# Autodesk Inventor assembly: Sistema movimiento izquierdo
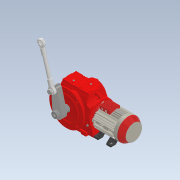
[picture p0: Inventor's stored thumbnail of the model, 180x180]
Saved by Autodesk Inventor 2021 (Build 250183000, 183)
## iProperties
Created: 2021-06-19
Part Number: Sistema movimiento izquierdo
Document SubType Name: Assembly
Designer: Andrés Holguín
Author: Andrés Holguín
## Documents named in this file (8)
- C:\Users\andre\Documents\GitHub\Dis.-Mecatronico-E6\inventor proyecto\Motores y reductores\Sistema movimiento izquierdo.iam
- C:\Users\andre\Documents\GitHub\Dis.-Mecatronico-E6\inventor proyecto\Motores y reductores\Reductor Izquierda.iam
- C:\Users\andre\Documents\GitHub\Dis.-Mecatronico-E6\inventor proyecto\Motores y reductores\placa manivela.ipt
- C:\Users\andre\Documents\GitHub\Dis.-Mecatronico-E6\inventor proyecto\Motores y reductores\pasador.ipt
- C:\Users\andre\Documents\GitHub\Dis.-Mecatronico-E6\inventor proyecto\Motores y reductores\Biela Completa.iam
- C:\Users\andre\Documents\GitHub\Dis.-Mecatronico-E6\inventor proyecto\Motores y reductores\Motor Simens Frame 112M IM B3.ipt
- C:\Users\andre\Documents\Inventor\Content Center Files\R2021\en-US\AS 1421(4)\AS 1421 - M16 x 16 Flat Point.ipt
- C:\Users\andre\Documents\Inventor\Content Center Files\R2021\en-US\AS 2465(3)\AS 2465 - 1  UNC(2).ipt
## Components (7 placed, 7 different names)
1. Reductor Izquierda:1 [sub-assembly] — Insert:3, Mate:1, Rigid:2
2. placa manivela:1 — Insert:3, Mate:1, Insert:4, Rigid:3
3. pasador:1 — Insert:4, Insert:5, Rotational:1
4. Motor Simens Frame 112M IM B3:1 — Rigid:2
5. Biela Completa:1 [sub-assembly] — Insert:5
6. AS 2465 (Unified hexagon bolts, screws and nuts (UNC and UNF threads) - Inch 1  UNC:1 — Rotational:1
7. AS 1421 Flat Point - Metric M16 x 16 Flat Point:1 — Rigid:3
## Relationships (7: Insert 3, WeldJoint 2, Mate 1, RevoluteJoint 1)
- Insert:3 (30 mm): Reductor Izquierda:1 ↔ placa manivela:1
- Mate:1: Reductor Izquierda:1 ↔ placa manivela:1
- Insert:4: placa manivela:1 ↔ pasador:1
- Rigid:2 [WeldJoint]: Reductor Izquierda:1 ↔ Motor Simens Frame 112M IM B3:1
- Insert:5 (20 mm): pasador:1 ↔ Biela Completa:1
- Rotational:1 [RevoluteJoint] (-2 mm): pasador:1 ↔ AS 2465 (Unified hexagon bolts, screws and nuts (UNC and UNF threads) - Inch 1  UNC:1
- Rigid:3 [WeldJoint]: placa manivela:1 ↔ AS 1421 Flat Point - Metric M16 x 16 Flat Point:1
